# Autodesk Inventor assembly: Flywheel
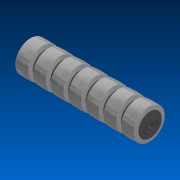
[picture p0: Inventor's stored thumbnail of the model, 180x180]
Saved by Autodesk Inventor 2022.2 (Build 262287000, 287)
## iProperties
Created: 2022-01-05
Part Number: Flywheel
Document SubType Name: Assembly
Designer: omard
Mass: 1051.35 g
Surface Area: 1523.99 cm^2
Volume: 930.396 cm^3
Density: 1.13 g/cm^3
Author: omard
## Documents named in this file (2)
- D:\omard\OneDrive - Auburn University\BasketBall Shooting Robot\Flywheel.iam
- D:\omard\OneDrive - Auburn University\BasketBall Shooting Robot\VEX Parts\Colson Performa 3 x 1.5, 1_2 Hex bore (217-4050).ipt
## Components (7 placed, 1 different names)
1. Colson Performa 3 x 1.5, 1_2 Hex bore (217-4050):1 — Flush:1, Flush:4, Mate:2, Mate:3, Mate:10, Mate:9, Mate:8
2. Colson Performa 3 x 1.5, 1_2 Hex bore (217-4050):2 — Flush:2, Flush:5, Mate:1, Mate:2
3. Colson Performa 3 x 1.5, 1_2 Hex bore (217-4050):3 — Flush:3, Flush:6, Mate:3, Angle:1, Angle:3, Mate:6, Mate:7
4. Colson Performa 3 x 1.5, 1_2 Hex bore (217-4050):4 — Flush:1, Flush:2, Flush:3, Flush:4, Flush:5, Flush:6, Mate:1, Angle:1, Angle:2, Mate:4, Mate:5
5. Colson Performa 3 x 1.5, 1_2 Hex bore (217-4050):5 — Angle:2, Mate:4, Mate:5
6. Colson Performa 3 x 1.5, 1_2 Hex bore (217-4050):6 — Angle:3, Mate:6, Mate:7, Mate:11, Angle:4, Mate:12
7. Colson Performa 3 x 1.5, 1_2 Hex bore (217-4050):7 — Mate:11, Angle:4, Mate:12
## Relationships (22: Mate 12, Flush 6, Angle 4)
- Flush:1: Colson Performa 3 x 1.5, 1_2 Hex bore (217-4050):1 ↔ Colson Performa 3 x 1.5, 1_2 Hex bore (217-4050):4
- Flush:2: Colson Performa 3 x 1.5, 1_2 Hex bore (217-4050):2 ↔ Colson Performa 3 x 1.5, 1_2 Hex bore (217-4050):4
- Flush:3: Colson Performa 3 x 1.5, 1_2 Hex bore (217-4050):3 ↔ Colson Performa 3 x 1.5, 1_2 Hex bore (217-4050):4
- Flush:4: Colson Performa 3 x 1.5, 1_2 Hex bore (217-4050):1 ↔ Colson Performa 3 x 1.5, 1_2 Hex bore (217-4050):4
- Flush:5: Colson Performa 3 x 1.5, 1_2 Hex bore (217-4050):2 ↔ Colson Performa 3 x 1.5, 1_2 Hex bore (217-4050):4
- Flush:6: Colson Performa 3 x 1.5, 1_2 Hex bore (217-4050):3 ↔ Colson Performa 3 x 1.5, 1_2 Hex bore (217-4050):4
- Mate:1: Colson Performa 3 x 1.5, 1_2 Hex bore (217-4050):2 ↔ Colson Performa 3 x 1.5, 1_2 Hex bore (217-4050):4
- Mate:2: Colson Performa 3 x 1.5, 1_2 Hex bore (217-4050):1 ↔ Colson Performa 3 x 1.5, 1_2 Hex bore (217-4050):2
- Mate:3: Colson Performa 3 x 1.5, 1_2 Hex bore (217-4050):1 ↔ Colson Performa 3 x 1.5, 1_2 Hex bore (217-4050):3
- Angle:1 (0 deg): Colson Performa 3 x 1.5, 1_2 Hex bore (217-4050):3 ↔ Colson Performa 3 x 1.5, 1_2 Hex bore (217-4050):4
- Angle:2 (0 deg): Colson Performa 3 x 1.5, 1_2 Hex bore (217-4050):4 ↔ Colson Performa 3 x 1.5, 1_2 Hex bore (217-4050):5
- Mate:4: Colson Performa 3 x 1.5, 1_2 Hex bore (217-4050):4 ↔ Colson Performa 3 x 1.5, 1_2 Hex bore (217-4050):5
- Mate:5: Colson Performa 3 x 1.5, 1_2 Hex bore (217-4050):4 ↔ Colson Performa 3 x 1.5, 1_2 Hex bore (217-4050):5
- Angle:3 (0 deg): Colson Performa 3 x 1.5, 1_2 Hex bore (217-4050):3 ↔ Colson Performa 3 x 1.5, 1_2 Hex bore (217-4050):6
- Mate:6: Colson Performa 3 x 1.5, 1_2 Hex bore (217-4050):3 ↔ Colson Performa 3 x 1.5, 1_2 Hex bore (217-4050):6
- Mate:7: Colson Performa 3 x 1.5, 1_2 Hex bore (217-4050):3 ↔ Colson Performa 3 x 1.5, 1_2 Hex bore (217-4050):6
- Mate:8: Colson Performa 3 x 1.5, 1_2 Hex bore (217-4050):1
- Mate:10: Colson Performa 3 x 1.5, 1_2 Hex bore (217-4050):1
- Mate:9: Colson Performa 3 x 1.5, 1_2 Hex bore (217-4050):1
- Mate:11: Colson Performa 3 x 1.5, 1_2 Hex bore (217-4050):6 ↔ Colson Performa 3 x 1.5, 1_2 Hex bore (217-4050):7
- Angle:4 (0 deg): Colson Performa 3 x 1.5, 1_2 Hex bore (217-4050):6 ↔ Colson Performa 3 x 1.5, 1_2 Hex bore (217-4050):7
- Mate:12: Colson Performa 3 x 1.5, 1_2 Hex bore (217-4050):6 ↔ Colson Performa 3 x 1.5, 1_2 Hex bore (217-4050):7
